# Autodesk Inventor assembly: WallEAssembly
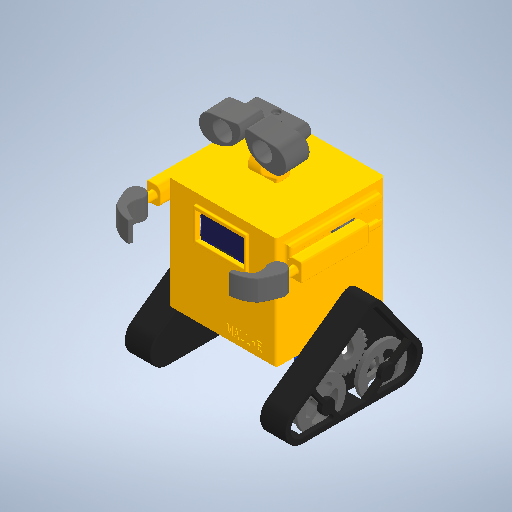
[picture p0: Inventor's stored thumbnail of the model, 512x512]
Saved by Autodesk Inventor 2025.2 (Build 292293000, 293)
## iProperties
Created: 2025-01-25
Part Number: WallEAssembly
Document SubType Name: Assembly
Designer: andre
Author: andre
## Documents named in this file (24)
- C:\Users\andre\Documents\GitHub\Handshake\Hardware\Proto2-WallE\WallEAssembly.iam
- C:\Users\andre\Documents\GitHub\Handshake\Hardware\Proto2-WallE\WallEBody.ipt
- C:\Users\andre\Documents\GitHub\Handshake\Hardware\Common\PCBModel.ipt
- C:\Users\andre\Documents\GitHub\Handshake\Hardware\Common\Battery_9V\Battery_9V\Battery_9V.ipt
- C:\Users\andre\Documents\GitHub\Handshake\Hardware\Proto2-WallE\TreadAssembly.iam
- C:\Users\andre\Documents\GitHub\Handshake\Hardware\Common\Servo Motor SG90.ipt
- C:\Users\andre\Documents\GitHub\Handshake\Hardware\Proto2-WallE\ BodyLid.ipt
- C:\Users\andre\Documents\GitHub\Handshake\Hardware\Proto2-WallE\WheelBetter.ipt
- C:\Users\andre\Documents\GitHub\Handshake\Hardware\Proto2-WallE\WallEAssembly\Design Accelerator\Spur Gear21.ipt
- C:\Users\andre\Documents\GitHub\Handshake\Hardware\Proto2-WallE\WallEAssembly\Design Accelerator\Spur Gear11.ipt
- C:\Users\andre\Documents\GitHub\Handshake\Hardware\Proto2-WallE\Arm.ipt
- C:\Users\andre\Documents\GitHub\Handshake\Hardware\Proto2-WallE\ArmLength.ipt
- C:\Users\andre\Documents\GitHub\Handshake\Hardware\Proto2-WallE\Hand.ipt
- C:\Users\andre\Documents\GitHub\Handshake\Hardware\Proto2-WallE\Neck.ipt
- C:\Users\andre\Documents\GitHub\Handshake\Hardware\Proto2-WallE\Eyes.ipt
- C:\Users\andre\Documents\GitHub\Handshake\Hardware\Common\Oled SH1106\Oled SH1106\Oled SH1106.ipt
- C:\Users\andre\Documents\GitHub\Handshake\Hardware\Proto2-WallE\TreadAssembly_MIR.iam
- C:\Users\andre\Documents\GitHub\Handshake\Hardware\Proto2-WallE\WheelBetter_MIR.ipt
- C:\Users\andre\Documents\GitHub\Handshake\Hardware\Proto2-WallE\WallEAssembly\Design Accelerator\Spur Gear21_MIR.ipt
- C:\Users\andre\Documents\GitHub\Handshake\Hardware\Proto2-WallE\WallEAssembly\Design Accelerator\Spur Gear11_MIR.ipt
- C:\Users\andre\Documents\GitHub\Handshake\Hardware\Proto2-WallE\Arm_MIR.ipt
- C:\Users\andre\Documents\GitHub\Handshake\Hardware\Proto2-WallE\ArmLength_MIR.ipt
- C:\Users\andre\Documents\GitHub\Handshake\Hardware\Proto2-WallE\Hand_MIR.ipt
- C:\Users\andre\Documents\GitHub\Handshake\Hardware\Proto2-WallE\BodyLid.ipt
## Components (23 placed, 22 different names)
1. WallEBody:1 — Mate:1, Angle:1, Mate:2, Mate:3, Mate:4, Angle:2, Mate:5, Mate:6, Mate:8, Mate:9, Flush:1, Flush:2, Mate:24, Mate:25, Angle:5, Mate:32, Mate:33, Mate:48, Mate:52, Mate:53, Mate:54, Mate:55, Mate:56
2. PCBModel:1 — Mate:1, Angle:1, Mate:2
3. Battery_9V:1 — Mate:3, Mate:8
4. TreadAssembly:1 [sub-assembly] — Mate:4, Angle:2, Mate:5, Mate:6, Mate:7, Mate:13, Mate:14, Mate:15, Mate:18, Mate:30
5. Servo Motor SG90:1 — Mate:7, Mate:9, Mate:13, Mate:16, Mate:17
6. BodyLid:1 — Flush:1, Flush:2, Mate:26, Mate:27
7. WheelBetter:1 — Mate:14, Mate:30
8. Spur Gear2:1 — Mate:16, Mate:17
9. Spur Gear1:1 — Mate:15, Mate:18
10. Arm:1 — Mate:19, Angle:3, Mate:22, Mate:23, Mate:24, Mate:25
11. ArmLength:1 — Mate:19, Angle:3, Mate:20, Mate:21, Mate:22, Mate:23
12. Hand:1 — Mate:20, Mate:21
13. Neck:1 — Mate:26, Mate:27, Angle:4, Mate:28, Mate:29
14. Eyes:1 — Angle:4, Mate:28, Mate:29
15. Oled SH1106:1 — Angle:5, Mate:32, Mate:33
16. TreadAssembly_MIR:1 [sub-assembly] — Mate:36, Mate:37, Mate:40, Mate:41, Mate:47, Mate:50, Mate:51, Mate:52, Mate:53, Mate:54
17. WheelBetter_MIR:1 — Mate:36, Mate:37
18. Spur Gear21_MIR:1 — Mate:49, Mate:50
19. Spur Gear11_MIR:1 — Mate:40, Mate:41
20. Arm_MIR:1 — Mate:42, Mate:43, Angle:6, Mate:44, Mate:55, Mate:56
21. ArmLength_MIR:1 — Mate:42, Mate:43, Angle:6, Mate:44, Mate:45, Mate:46
22. Hand_MIR:1 — Mate:45, Mate:46
23. Servo Motor SG90:2 — Mate:47, Mate:48, Mate:49, Mate:51
## Relationships (56: Mate 48, Angle 6, Flush 2)
- Mate:1 (2.3 mm): WallEBody:1 ↔ PCBModel:1
- Angle:1 (0 deg): WallEBody:1 ↔ PCBModel:1
- Mate:2: WallEBody:1 ↔ PCBModel:1
- Mate:3: WallEBody:1 ↔ Battery_9V:1
- Mate:4: WallEBody:1 ↔ TreadAssembly:1
- Angle:2 (0 deg): WallEBody:1 ↔ TreadAssembly:1
- Mate:5: WallEBody:1 ↔ TreadAssembly:1
- Mate:6: WallEBody:1 ↔ TreadAssembly:1
- Mate:7: TreadAssembly:1 ↔ Servo Motor SG90:1
- Mate:8: WallEBody:1 ↔ Battery_9V:1
- Mate:9: WallEBody:1 ↔ Servo Motor SG90:1
- Flush:1: WallEBody:1 ↔ BodyLid:1
- Flush:2: WallEBody:1 ↔ BodyLid:1
- Mate:13: TreadAssembly:1 ↔ Servo Motor SG90:1
- Mate:14: TreadAssembly:1 ↔ WheelBetter:1
- Mate:15: TreadAssembly:1 ↔ Spur Gear1:1
- Mate:16: Servo Motor SG90:1 ↔ Spur Gear2:1
- Mate:17: Servo Motor SG90:1 ↔ Spur Gear2:1
- Mate:18: TreadAssembly:1 ↔ Spur Gear1:1
- Mate:19: Arm:1 ↔ ArmLength:1
- Angle:3 (0 deg): Arm:1 ↔ ArmLength:1
- Mate:20: ArmLength:1 ↔ Hand:1
- Mate:21: ArmLength:1 ↔ Hand:1
- Mate:22: Arm:1 ↔ ArmLength:1
- Mate:23: Arm:1 ↔ ArmLength:1
- Mate:24: WallEBody:1 ↔ Arm:1
- Mate:25: WallEBody:1 ↔ Arm:1
- Mate:26: BodyLid:1 ↔ Neck:1
- Mate:27: BodyLid:1 ↔ Neck:1
- Angle:4 (90 deg): Neck:1 ↔ Eyes:1
- Mate:28: Neck:1 ↔ Eyes:1
- Mate:29: Neck:1 ↔ Eyes:1
- Mate:30: TreadAssembly:1 ↔ WheelBetter:1
- Angle:5 (0 deg): WallEBody:1 ↔ Oled SH1106:1
- Mate:32: WallEBody:1 ↔ Oled SH1106:1
- Mate:33: WallEBody:1 ↔ Oled SH1106:1
- Mate:36: TreadAssembly_MIR:1 ↔ WheelBetter_MIR:1
- Mate:37: TreadAssembly_MIR:1 ↔ WheelBetter_MIR:1
- Mate:40: TreadAssembly_MIR:1 ↔ Spur Gear11_MIR:1
- Mate:41: TreadAssembly_MIR:1 ↔ Spur Gear11_MIR:1
- Mate:42: Arm_MIR:1 ↔ ArmLength_MIR:1
- Mate:43: Arm_MIR:1 ↔ ArmLength_MIR:1
- Angle:6 (0 deg): Arm_MIR:1 ↔ ArmLength_MIR:1
- Mate:44: Arm_MIR:1 ↔ ArmLength_MIR:1
- Mate:45: ArmLength_MIR:1 ↔ Hand_MIR:1
- Mate:46: ArmLength_MIR:1 ↔ Hand_MIR:1
- Mate:47: TreadAssembly_MIR:1 ↔ Servo Motor SG90:2
- Mate:48: WallEBody:1 ↔ Servo Motor SG90:2
- Mate:49: Spur Gear21_MIR:1 ↔ Servo Motor SG90:2
- Mate:50: TreadAssembly_MIR:1 ↔ Spur Gear21_MIR:1
- Mate:51: TreadAssembly_MIR:1 ↔ Servo Motor SG90:2
- Mate:52: WallEBody:1 ↔ TreadAssembly_MIR:1
- Mate:53: WallEBody:1 ↔ TreadAssembly_MIR:1
- Mate:54: WallEBody:1 ↔ TreadAssembly_MIR:1
- Mate:55: WallEBody:1 ↔ Arm_MIR:1
- Mate:56: WallEBody:1 ↔ Arm_MIR:1
